# Autodesk Inventor assembly: KillSwitchAssembly
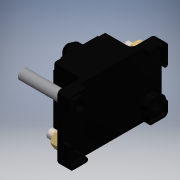
[picture p0: Inventor's stored thumbnail of the model, 180x180]
Saved by Autodesk Inventor 2017 (Build 210142000, 142)
## iProperties
Created: 2020-02-29
Part Number: KillSwitchAssembly
Document SubType Name: Assembly
Designer: S338674153
Author: S338674153
## Documents named in this file (3)
- \\ad.ocdsb.ca\studenthome\3\S338674153\FRC 2020\FullRobotRefactor\Parts\KillSwitchAssembly.iam
- \\ad.ocdsb.ca\studenthome\3\S338674153\FRC 2020\FullRobotRefactor\Parts\am-0282 120a Circuit Breaker.ipt
- \\ad.ocdsb.ca\studenthome\3\S338674153\FRC 2020\FullRobotRefactor\Parts\KillSwitchStandoff.ipt
## Components (3 placed, 2 different names)
1. am-0282 120a Circuit Breaker:1 — Mate:2, Mate:3, Mate:4, Mate:5
2. KillSwitchStandoff:1 — Mate:2, Mate:5
3. KillSwitchStandoff:2 — Mate:3, Mate:4
## Relationships (4: Mate 4)
- Mate:2: am-0282 120a Circuit Breaker:1 ↔ KillSwitchStandoff:1
- Mate:3: am-0282 120a Circuit Breaker:1 ↔ KillSwitchStandoff:2
- Mate:4: am-0282 120a Circuit Breaker:1 ↔ KillSwitchStandoff:2
- Mate:5: am-0282 120a Circuit Breaker:1 ↔ KillSwitchStandoff:1
